# Autodesk Inventor assembly: SecondJoint
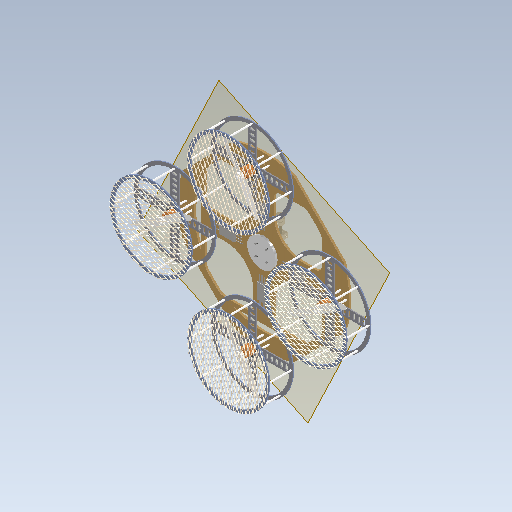
[picture p0: Inventor's stored thumbnail of the model, 512x512]
Saved by Autodesk Inventor 2021.1 (Build 251245010, 245A)
## iProperties
Created: 2023-10-17
Part Number: SecondJoint
Document SubType Name: Assembly
Designer: Lenovo
Mass: 2023.96 g
Surface Area: 8827.15 cm^2
Volume: 1258.18 cm^3
Density: 1.60864 g/cm^3
Author: Lenovo
## Documents named in this file (13)
- F:\College\Semester_10\GP2\2DOF\2DOF_Hover\CAD\Workspaces\Workspace\SecondJoint.iam
- F:\College\Semester_10\GP2\2DOF\2DOF_Hover\CAD\Workspaces\Workspace\Assembly231015Kerangka Bawah 1.ipt
- F:\College\Semester_10\GP2\2DOF\2DOF_Hover\CAD\Workspaces\Workspace\shaft.ipt
- F:\College\Semester_10\GP2\2DOF\2DOF_Hover\CAD\Workspaces\Workspace\SK8.ipt
- F:\College\Semester_10\GP2\2DOF\2DOF_Hover\CAD\Workspaces\Workspace\Part15.ipt
- F:\College\Semester_10\GP2\2DOF\2DOF_Hover\CAD\Workspaces\Workspace\Assembly1.iam
- F:\College\Semester_10\GP2\2DOF\2DOF_Hover\CAD\Workspaces\Workspace\Libraries\Content Center Files\en-US\BS EN ISO 4015\BS EN ISO 4015 - M3x20.ipt
- F:\College\Semester_10\GP2\2DOF\2DOF_Hover\CAD\Workspaces\Workspace\Libraries\Content Center Files\en-US\AS 1112 (4)\AS 1112 - M3(2).ipt
- F:\College\Semester_10\GP2\2DOF\2DOF_Hover\CAD\Workspaces\Workspace\Libraries\Content Center Files\en-US\ISO 4034(2)\ISO 4034 - M5 - ISO.ipt
- F:\College\Semester_10\GP2\2DOF\2DOF_Hover\CAD\Libraries\Content Center Files\en-US\ISO 4015\ISO 4015 - M5 x 45.ipt
- F:\College\Semester_10\GP2\2DOF\2DOF_Hover\CAD\Workspaces\Workspace\pcb.ipt
- F:\College\Semester_10\GP2\2DOF\2DOF_Hover\CAD\Workspaces\Workspace\Esc_BlHeli_30A.ipt
- F:\College\Semester_10\GP2\2DOF\2DOF_Hover\CAD\Workspaces\Workspace\Coupler_5x8.ipt
## Components (43 placed, 12 different names)
1. Kerangka Bawah 1_10 — Flush:2, Flush:3, Mate:55, Mate:56, Mate:57, Mate:79, Mate:82, Mate:85, Mate:88, Insert:1, Insert:2, Insert:3, Insert:4, Insert:5, Insert:6, Insert:7, Insert:8, Insert:9, Insert:10, Insert:11, Insert:12, Insert:13, Insert:14, Insert:15, Insert:16, Angle:2, Angle:3, Angle:4, Angle:5, Angle:6, Angle:7, Angle:8, Angle:9, Angle:10, Angle:11, Angle:12, Angle:13, Angle:14, Angle:15, Angle:16, Angle:17, Insert:21, Mate:111, Mate:112, Mate:113, Flush:6, Flush:7, Mate:122, Mate:127, Mate:129, Mate:131, Mate:133, Mate:137, Flush:8, Flush:9, Mate:138, Mate:139, Mate:140, Flush:10, Flush:11, Flush:12, Flush:13, Flush:14, Flush:15
2. SK8:1 — Mate:50, Mate:54, Mate:98, Mate:99, Angle:19, Mate:100, Mate:101, Mate:109, Mate:110, Mate:123, Mate:134, Mate:136
3. SK8:2 — Angle:1, Mate:47, Mate:53, Angle:22, Mate:102, Mate:103, Mate:105, Mate:106, Mate:107, Mate:108, Mate:135
4. shaft:1 — Angle:1, Mate:53, Mate:54, Mate:123, Mate:141, Mate:142
5. Part15:1 — Flush:2, Flush:3, Mate:47, Mate:50, Mate:55, Mate:56, Mate:57, Mate:100, Mate:101, Mate:102, Mate:103
6. pcb:1 — Flush:6, Flush:7, Mate:122
7. Coupler_5x8:1 — Mate:141, Mate:142
8. Assembly1:1 [sub-assembly] — Mate:79, Insert:17, Insert:18, Insert:19, Insert:20, Mate:126, Mate:127
9. Assembly1:2 [sub-assembly] — Mate:85, Mate:128, Mate:129
10. Assembly1:3 [sub-assembly] — Mate:88, Mate:130, Mate:131
11. Assembly1:4 [sub-assembly] — Mate:82, Mate:132, Mate:133
12. ISO 4015 M5 x 45:2 — Mate:105, Mate:106, Mate:115
13. ISO 4034 M5:2 — Mate:111, Mate:114
14. ISO 4015 M5 x 45:3 — Mate:107, Mate:108, Mate:116
15. ISO 4034 M5:3 — Mate:112, Mate:115
16. ISO 4015 M5 x 45:4 — Mate:109, Mate:110, Mate:114
17. ISO 4034 M5:4 — Mate:113, Mate:116
18. BS EN ISO 4015 M3x20:1 — Insert:1, Angle:2, Mate:126
19. BS EN ISO 4015 M3x20:2 — Insert:2, Angle:15
20. BS EN ISO 4015 M3x20:3 — Insert:3, Angle:4
21. BS EN ISO 4015 M3x20:4 — Insert:4, Angle:6
22. BS EN ISO 4015 M3x20:5 — Insert:5, Angle:12
23. BS EN ISO 4015 M3x20:6 — Insert:6, Angle:13
24. BS EN ISO 4015 M3x20:7 — Insert:7, Angle:7
25. BS EN ISO 4015 M3x20:8 — Insert:8, Angle:14
26. BS EN ISO 4015 M3x20:9 — Insert:9, Angle:17, Mate:128
27. BS EN ISO 4015 M3x20:10 — Insert:10, Angle:3
28. BS EN ISO 4015 M3x20:11 — Insert:11, Angle:8
29. BS EN ISO 4015 M3x20:12 — Insert:12, Angle:11
30. BS EN ISO 4015 M3x20:13 — Insert:13, Angle:10, Mate:130
31. BS EN ISO 4015 M3x20:14 — Insert:14, Angle:9, Mate:132
32. BS EN ISO 4015 M3x20:15 — Insert:15, Angle:5
33. BS EN ISO 4015 M3x20:16 — Insert:16, Angle:16
34. AS 1112 (4) - Metric M3:1 — Insert:17
35. AS 1112 (4) - Metric M3:2 — Insert:18
36. AS 1112 (4) - Metric M3:3 — Insert:19
37. AS 1112 (4) - Metric M3:4 — Insert:20
38. ISO 4015 M5 x 45:1 — Mate:98, Mate:99, Angle:19
39. ISO 4034 M5:1 — Insert:21, Angle:22
40. Esc_BlHeli_30A:1 — Mate:137, Flush:8, Flush:9
41. Esc_BlHeli_30A:2 — Mate:138, Flush:10, Flush:11
42. Esc_BlHeli_30A:3 — Mate:139, Flush:12, Flush:13
43. Esc_BlHeli_30A:4 — Mate:140, Flush:14, Flush:15
## Relationships (100: Mate 48, Insert 21, Angle 19, Flush 12)
- Angle:1 (0 deg): SK8:2 ↔ shaft:1
- Flush:2: Kerangka Bawah 1_10 ↔ Part15:1
- Flush:3: Kerangka Bawah 1_10 ↔ Part15:1
- Mate:47: SK8:2 ↔ Part15:1
- Mate:50: SK8:1 ↔ Part15:1
- Mate:53: SK8:2 ↔ shaft:1
- Mate:54: SK8:1 ↔ shaft:1
- Mate:55: Kerangka Bawah 1_10 ↔ Part15:1
- Mate:56: Kerangka Bawah 1_10 ↔ Part15:1
- Mate:57: Kerangka Bawah 1_10 ↔ Part15:1
- Mate:79: Kerangka Bawah 1_10 ↔ Assembly1:1
- Mate:82: Kerangka Bawah 1_10 ↔ Assembly1:4
- Mate:85: Kerangka Bawah 1_10 ↔ Assembly1:2
- Mate:88: Kerangka Bawah 1_10 ↔ Assembly1:3
- Insert:1: Kerangka Bawah 1_10 ↔ BS EN ISO 4015 M3x20:1
- Insert:2: Kerangka Bawah 1_10 ↔ BS EN ISO 4015 M3x20:2
- Insert:3: Kerangka Bawah 1_10 ↔ BS EN ISO 4015 M3x20:3
- Insert:4: Kerangka Bawah 1_10 ↔ BS EN ISO 4015 M3x20:4
- Insert:5: Kerangka Bawah 1_10 ↔ BS EN ISO 4015 M3x20:5
- Insert:6: Kerangka Bawah 1_10 ↔ BS EN ISO 4015 M3x20:6
- Insert:7: Kerangka Bawah 1_10 ↔ BS EN ISO 4015 M3x20:7
- Insert:8: Kerangka Bawah 1_10 ↔ BS EN ISO 4015 M3x20:8
- Insert:9: Kerangka Bawah 1_10 ↔ BS EN ISO 4015 M3x20:9
- Insert:10: Kerangka Bawah 1_10 ↔ BS EN ISO 4015 M3x20:10
- Insert:11: Kerangka Bawah 1_10 ↔ BS EN ISO 4015 M3x20:11
- Insert:12: Kerangka Bawah 1_10 ↔ BS EN ISO 4015 M3x20:12
- Insert:13: Kerangka Bawah 1_10 ↔ BS EN ISO 4015 M3x20:13
- Insert:14: Kerangka Bawah 1_10 ↔ BS EN ISO 4015 M3x20:14
- Insert:15: Kerangka Bawah 1_10 ↔ BS EN ISO 4015 M3x20:15
- Insert:16: Kerangka Bawah 1_10 ↔ BS EN ISO 4015 M3x20:16
- Insert:17: Assembly1:1 ↔ AS 1112 (4) - Metric M3:1
- Insert:18: Assembly1:1 ↔ AS 1112 (4) - Metric M3:2
- Insert:19: Assembly1:1 ↔ AS 1112 (4) - Metric M3:3
- Insert:20: Assembly1:1 ↔ AS 1112 (4) - Metric M3:4
- Angle:2 (0 deg): Kerangka Bawah 1_10 ↔ BS EN ISO 4015 M3x20:1
- Angle:3 (0 deg): Kerangka Bawah 1_10 ↔ BS EN ISO 4015 M3x20:10
- Angle:4 (0 deg): Kerangka Bawah 1_10 ↔ BS EN ISO 4015 M3x20:3
- Angle:5 (0 deg): Kerangka Bawah 1_10 ↔ BS EN ISO 4015 M3x20:15
- Angle:6 (0 deg): Kerangka Bawah 1_10 ↔ BS EN ISO 4015 M3x20:4
- Angle:7 (0 deg): Kerangka Bawah 1_10 ↔ BS EN ISO 4015 M3x20:7
- Angle:8 (0 deg): Kerangka Bawah 1_10 ↔ BS EN ISO 4015 M3x20:11
- Angle:9 (0 deg): Kerangka Bawah 1_10 ↔ BS EN ISO 4015 M3x20:14
- Angle:10 (0 deg): Kerangka Bawah 1_10 ↔ BS EN ISO 4015 M3x20:13
- Angle:11 (0 deg): Kerangka Bawah 1_10 ↔ BS EN ISO 4015 M3x20:12
- Angle:12 (0 deg): Kerangka Bawah 1_10 ↔ BS EN ISO 4015 M3x20:5
- Angle:13 (0 deg): Kerangka Bawah 1_10 ↔ BS EN ISO 4015 M3x20:6
- Angle:14 (0 deg): Kerangka Bawah 1_10 ↔ BS EN ISO 4015 M3x20:8
- Angle:15 (0 deg): Kerangka Bawah 1_10 ↔ BS EN ISO 4015 M3x20:2
- Angle:16 (0 deg): Kerangka Bawah 1_10 ↔ BS EN ISO 4015 M3x20:16
- Angle:17 (0 deg): Kerangka Bawah 1_10 ↔ BS EN ISO 4015 M3x20:9
- Mate:98: SK8:1 ↔ ISO 4015 M5 x 45:1
- Mate:99: SK8:1 ↔ ISO 4015 M5 x 45:1
- Angle:19 (0 deg): SK8:1 ↔ ISO 4015 M5 x 45:1
- Insert:21: Kerangka Bawah 1_10 ↔ ISO 4034 M5:1
- Angle:22 (0 deg): SK8:2 ↔ ISO 4034 M5:1
- Mate:100: SK8:1 ↔ Part15:1
- Mate:101: SK8:1 ↔ Part15:1
- Mate:102: SK8:2 ↔ Part15:1
- Mate:103: SK8:2 ↔ Part15:1
- Mate:105: SK8:2 ↔ ISO 4015 M5 x 45:2
- Mate:106: SK8:2 ↔ ISO 4015 M5 x 45:2
- Mate:107: SK8:2 ↔ ISO 4015 M5 x 45:3
- Mate:108: SK8:2 ↔ ISO 4015 M5 x 45:3
- Mate:109: SK8:1 ↔ ISO 4015 M5 x 45:4
- Mate:110: SK8:1 ↔ ISO 4015 M5 x 45:4
- Mate:111: Kerangka Bawah 1_10 ↔ ISO 4034 M5:2
- Mate:112: Kerangka Bawah 1_10 ↔ ISO 4034 M5:3
- Mate:113: Kerangka Bawah 1_10 ↔ ISO 4034 M5:4
- Mate:114: ISO 4034 M5:2 ↔ ISO 4015 M5 x 45:4
- Mate:115: ISO 4015 M5 x 45:2 ↔ ISO 4034 M5:3
- Mate:116: ISO 4015 M5 x 45:3 ↔ ISO 4034 M5:4
- Flush:6: Kerangka Bawah 1_10 ↔ pcb:1
- Flush:7: Kerangka Bawah 1_10 ↔ pcb:1
- Mate:122: Kerangka Bawah 1_10 ↔ pcb:1
- Mate:123 (-48 mm): SK8:1 ↔ shaft:1
- Mate:126: Assembly1:1 ↔ BS EN ISO 4015 M3x20:1
- Mate:127: Kerangka Bawah 1_10 ↔ Assembly1:1
- Mate:128: Assembly1:2 ↔ BS EN ISO 4015 M3x20:9
- Mate:129: Kerangka Bawah 1_10 ↔ Assembly1:2
- Mate:130: Assembly1:3 ↔ BS EN ISO 4015 M3x20:13
- Mate:131: Kerangka Bawah 1_10 ↔ Assembly1:3
- Mate:132: Assembly1:4 ↔ BS EN ISO 4015 M3x20:14
- Mate:133: Kerangka Bawah 1_10 ↔ Assembly1:4
- Mate:134: SK8:1
- Mate:135 (-9 mm): SK8:2
- Mate:136 (-23 mm): SK8:1
- Mate:137: Kerangka Bawah 1_10 ↔ Esc_BlHeli_30A:1
- Flush:8 (-60 mm): Kerangka Bawah 1_10 ↔ Esc_BlHeli_30A:1
- Flush:9 (17 mm): Kerangka Bawah 1_10 ↔ Esc_BlHeli_30A:1
- Mate:138: Kerangka Bawah 1_10 ↔ Esc_BlHeli_30A:2
- Mate:139: Kerangka Bawah 1_10 ↔ Esc_BlHeli_30A:3
- Mate:140: Kerangka Bawah 1_10 ↔ Esc_BlHeli_30A:4
- Flush:10 (60 mm): Kerangka Bawah 1_10 ↔ Esc_BlHeli_30A:2
- Flush:11 (17 mm): Kerangka Bawah 1_10 ↔ Esc_BlHeli_30A:2
- Flush:12 (60 mm): Kerangka Bawah 1_10 ↔ Esc_BlHeli_30A:3
- Flush:13 (17 mm): Kerangka Bawah 1_10 ↔ Esc_BlHeli_30A:3
- Flush:14 (60 mm): Kerangka Bawah 1_10 ↔ Esc_BlHeli_30A:4
- Flush:15 (17 mm): Kerangka Bawah 1_10 ↔ Esc_BlHeli_30A:4
- Mate:141: shaft:1 ↔ Coupler_5x8:1
- Mate:142 (-13 mm): shaft:1 ↔ Coupler_5x8:1
